# Autodesk Inventor assembly: Kirigami Bed
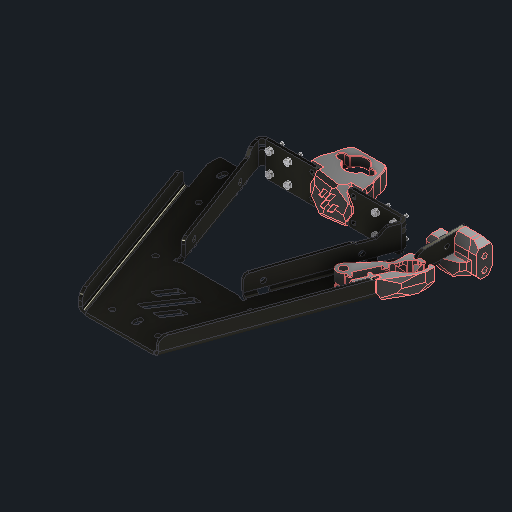
[picture p0: Inventor's stored thumbnail of the model, 512x512]
Saved by Autodesk Inventor 2025.1 (Build 291241020, 241B)
## iProperties
Created: 2025-05-10
Part Number: Kirigami Bed
Document SubType Name: Assembly
Designer: Joshua Eah
Author: Joshua Eah
## Documents named in this file (7)
- C:\Users\Joshua Eah\Documents\Voron 0.2\CAD\Master Assembly\Z Axis\Bed Assembly\Kirigami Bed.iam
- C:\Users\Joshua Eah\Documents\Voron 0.2\CAD\Master Assembly\Z Axis\Bed Assembly\Kirigami Bed.ipt
- C:\Users\Joshua Eah\Documents\Voron 0.2\CAD\Master Assembly\Z Axis\Bed Assembly\Nut Block.ipt
- C:\Users\Joshua Eah\Documents\Voron 0.2\CAD\Master Assembly\Z Axis\Bed Assembly\Wire Guide.ipt
- C:\Users\Joshua Eah\Documents\Voron 0.2\CAD\Master Assembly\Z Axis\Bed Assembly\Chain Mount.ipt
- C:\Users\Joshua Eah\Documents\Voron 0.2\CAD\Master Assembly\Z Axis\Bed Assembly\Chain Spacer.ipt
- C:\Users\Joshua Eah\Documents\Voron 0.2\CAD\Master Assembly\Hardware\M2x8 SHCS.ipt
## Components (13 placed, 6 different names)
1. Kirigami Bed:1 — Insert:1, Angle:1, Insert:2, Insert:3, Insert:4, Insert:5, Insert:8, Insert:9, Insert:10, Insert:11, Insert:12, Insert:13, Insert:14, Insert:15
2. Nut Block:1 — Insert:2, Insert:3
3. Wire Guide:1 — Insert:1, Angle:1
4. Chain Mount:1 — Insert:4, Insert:5, Insert:6, Insert:7
5. Chain Spacer:1 — Insert:6, Insert:7
6. M2x8 SHCS:1 — Insert:8
7. M2x8 SHCS:2 — Insert:9
8. M2x8 SHCS:3 — Insert:10
9. M2x8 SHCS:4 — Insert:11
10. M2x8 SHCS:5 — Insert:13
11. M2x8 SHCS:6 — Insert:12
12. M2x8 SHCS:7 — Insert:15
13. M2x8 SHCS:8 — Insert:14
## Relationships (16: Insert 15, Angle 1)
- Insert:1: Kirigami Bed:1 ↔ Wire Guide:1
- Angle:1 (0 deg): Kirigami Bed:1 ↔ Wire Guide:1
- Insert:2: Kirigami Bed:1 ↔ Nut Block:1
- Insert:3: Kirigami Bed:1 ↔ Nut Block:1
- Insert:4: Kirigami Bed:1 ↔ Chain Mount:1
- Insert:5: Kirigami Bed:1 ↔ Chain Mount:1
- Insert:6: Chain Mount:1 ↔ Chain Spacer:1
- Insert:7: Chain Mount:1 ↔ Chain Spacer:1
- Insert:8: Kirigami Bed:1 ↔ M2x8 SHCS:1
- Insert:9: Kirigami Bed:1 ↔ M2x8 SHCS:2
- Insert:10: Kirigami Bed:1 ↔ M2x8 SHCS:3
- Insert:11: Kirigami Bed:1 ↔ M2x8 SHCS:4
- Insert:12: Kirigami Bed:1 ↔ M2x8 SHCS:6
- Insert:13: Kirigami Bed:1 ↔ M2x8 SHCS:5
- Insert:14: Kirigami Bed:1 ↔ M2x8 SHCS:8
- Insert:15: Kirigami Bed:1 ↔ M2x8 SHCS:7
